# Autodesk Inventor assembly: ASSY,ROBOT,2026
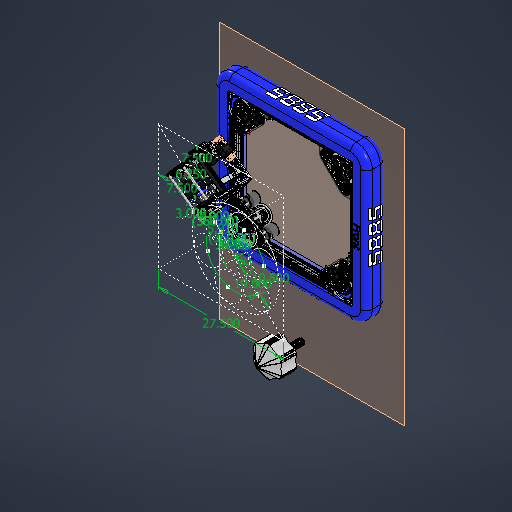
[picture p0: Inventor's stored thumbnail of the model, 512x512]
Saved by Autodesk Inventor 2026 (Build 300175000, 175)
## iProperties
Created: 2026-01-24
Part Number: ASSY,ROBOT,2026
Document SubType Name: Assembly
Designer: Jthib
Mass: 24729.3 g
Surface Area: 49621.3 cm^2
Volume: 29693.7 cm^3
Density: 0.832814 g/cm^3
Author: Jthib
## Documents named in this file (5)
- C:\Users\littl\OneDrive\Documents\GitHub\2026-Robot-Mechanical\ASSY,ROBOT,2026.iam
- C:\Users\littl\OneDrive\Documents\GitHub\2026-Robot-Mechanical\Chassis\CHASSIS.iam
- C:\Users\littl\OneDrive\Documents\GitHub\2026-Robot-Mechanical\Chassis\Bumpers.ipt
- C:\Users\littl\OneDrive\Documents\GitHub\2026-Robot-Mechanical\Spindexer\#Spindexer.iam
- C:\Users\littl\OneDrive\Documents\GitHub\2026-Robot-Mechanical\Shooter\Shooter - Front Motors\#SHOOTER.FRONT_MOTORS.iam
## Components (4 placed, 4 different names)
1. CHASSIS:1 [sub-assembly] — Flush:1, Flush:2, Flush:3, Flush:4, Mate:1, Mate:2, Mate:3, Mate:4, Mate:5
2. Bumpers:1 — Flush:4, Mate:1, Mate:2
3. #Spindexer:1 [sub-assembly]
4. #SHOOTER.FRONT_MOTORS:1 [sub-assembly] — Mate:3, Mate:4, Mate:5
## Relationships (9: Mate 5, Flush 4)
- Flush:1 (-349.25 mm): CHASSIS:1
- Flush:2 (349.25 mm): CHASSIS:1
- Flush:3: CHASSIS:1
- Flush:4 (-12.7 mm): CHASSIS:1 ↔ Bumpers:1
- Mate:1: CHASSIS:1 ↔ Bumpers:1
- Mate:2: CHASSIS:1 ↔ Bumpers:1
- Mate:3 (228.6 mm): CHASSIS:1 ↔ #SHOOTER.FRONT_MOTORS:1
- Mate:4 (-190.5 mm): CHASSIS:1 ↔ #SHOOTER.FRONT_MOTORS:1
- Mate:5 (-190.5 mm): CHASSIS:1 ↔ #SHOOTER.FRONT_MOTORS:1
